# Autodesk Inventor assembly: robot_1_13
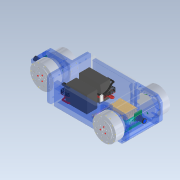
[picture p0: Inventor's stored thumbnail of the model, 180x180]
Saved by Autodesk Inventor 2020 (Build 240168000, 168)
## iProperties
Created: 2021-01-14
Part Number: robot_1_13
Document SubType Name: Assembly
Designer: DELL
Author: DELL
## Documents named in this file (19)
- F:\SoftRobot2.0\FlexipodHardware2.0\FlexipodHardware\Flexipod2.0\robot_2021_1_31\robot.iam
- F:\SoftRobot2.0\FlexipodHardware2.0\FlexipodHardware\Flexipod2.0\RMD_X6_stator.ipt
- F:\SoftRobot2.0\FlexipodHardware2.0\FlexipodHardware\Flexipod2.0\RMD_X6_rotor.ipt
- F:\SoftRobot2.0\FlexipodHardware2.0\FlexipodHardware\Flexipod2.0\Jetson nano v2- Inventor\Jetson_Nano_Dev_Kit_3D_b01.iam
- F:\SoftRobot2.0\FlexipodHardware2.0\FlexipodHardware\Flexipod2.0\battery_6s_1550_ovonic.ipt
- F:\SoftRobot2.0\FlexipodHardware2.0\FlexipodHardware\Flexipod2.0\Arducam Camera.ipt
- F:\SoftRobot2.0\FlexipodHardware2.0\FlexipodHardware\Flexipod2.0\robot_2021_1_27\shank_thigh_connector.ipt
- F:\SoftRobot2.0\FlexipodHardware2.0\FlexipodHardware\Flexipod2.0\robot_2021_1_28\hip_link_front.ipt
- F:\SoftRobot2.0\FlexipodHardware2.0\FlexipodHardware\Flexipod2.0\robot_2021_1_28\thigh_link.ipt
- F:\SoftRobot2.0\FlexipodHardware2.0\FlexipodHardware\Flexipod2.0\robot_2021_1_28\thigh_link_mirror.ipt
- F:\SoftRobot2.0\FlexipodHardware2.0\FlexipodHardware\Flexipod2.0\robot_2021_1_28\hip_link_front_mirror.ipt
- F:\SoftRobot2.0\FlexipodHardware2.0\FlexipodHardware\Flexipod2.0\robot_2021_1_28\shank_link_2.ipt
- F:\SoftRobot2.0\FlexipodHardware2.0\FlexipodHardware\Flexipod2.0\robot_2021_1_28\hip_back_motor_protector.ipt
- F:\SoftRobot2.0\FlexipodHardware2.0\FlexipodHardware\Flexipod2.0\robot_2021_1_28\hard_back_hip_2.ipt
- F:\SoftRobot2.0\FlexipodHardware2.0\FlexipodHardware\Flexipod2.0\robot_2021_1_28\hard_back_hip_2_mirror.ipt
- F:\SoftRobot2.0\FlexipodHardware2.0\FlexipodHardware\Flexipod2.0\robot_2021_1_31\back_motor_fix_board.ipt
- F:\SoftRobot2.0\FlexipodHardware2.0\FlexipodHardware\Flexipod2.0\robot_2021_1_31\buttom_camera_fix.ipt
- F:\SoftRobot2.0\FlexipodHardware2.0\FlexipodHardware\Flexipod2.0\robot_2021_1_28\body_soft2.ipt
- F:\SoftRobot2.0\FlexipodHardware2.0\FlexipodHardware\Flexipod2.0\robot_2021_1_28\body_soft2_2.ipt
## Components (55 placed, 18 different names)
1. RMD_X6_stator:1 — Mate:1, Flush:4, Mate:251, Mate:298, Mate:299
2. RMD_X6_rotor:1 — Mate:1, Flush:4, Mate:252, Mate:253
3. RMD_X6_stator:2 — Angle:2, Mate:254, Mate:255, Mate:256, Mate:257
4. RMD_X6_rotor:2 — Mate:247, Mate:248
5. RMD_X6_stator:3 — Mate:19, Mate:244, Mate:245, Mate:246
6. RMD_X6_rotor:3 — Mate:18, Mate:20
7. shank_thigh_connector:9 — Mate:18, Mate:19, Mate:20, Mate:262, Mate:263
8. RMD_X6_stator:4 — Mate:284, Mate:289, Mate:291
9. RMD_X6_rotor:4 — Mate:283, Mate:285
10. RMD_X6_stator:6 — Mate:44, Mate:231, Mate:232, Mate:233
11. RMD_X6_rotor:6 — Mate:42, Mate:43
12. shank_thigh_connector:10 — Mate:42, Mate:43, Mate:44, Mate:260, Mate:261
13. RMD_X6_rotor:7 — Flush:11, Mate:52, Mate:223, Mate:225
14. RMD_X6_stator:7 — Flush:11, Mate:52, Mate:56, Mate:57, Mate:58, Mate:224
15. RMD_X6_rotor:8 — Mate:51, Flush:10, Mate:53, Mate:54
16. RMD_X6_stator:8 — Mate:51, Flush:10, Mate:55, Mate:297, Mate:300
17. hip_link_front:1 — Mate:53, Mate:54, Mate:55, Mate:56, Mate:57, Mate:58
18. RMD_X6_rotor:9 — Mate:72, Mate:73
19. RMD_X6_stator:9 — Mate:74, Mate:228, Mate:229, Mate:230
20. RMD_X6_rotor:10 — Mate:276, Mate:278
21. RMD_X6_stator:10 — Mate:277, Mate:290, Mate:292
22. shank_thigh_connector:11 — Mate:72, Mate:73, Mate:74, Mate:264, Mate:265
23. Jetson_Nano_Dev_Kit_3D_b01:1 [sub-assembly]
24. battery_6s_1550_ovonic:1
25. battery_6s_1550_ovonic:2
26. Arducam Camera:1
27. Arducam Camera:2 — Angle:13, Mate:295, Flush:30
28. shank_link_2:3 — Mate:262, Mate:263
29. shank_link_2:4 — Mate:264, Mate:265
30. shank_link_2:2 — Mate:260, Mate:261
31. RMD_X6_rotor:13
32. RMD_X6_stator:13 — Mate:219, Mate:220, Mate:221
33. shank_thigh_connector:13 — Mate:258, Mate:259
34. shank_link_2:1 — Mate:258, Mate:259
35. RMD_X6_rotor:16 — Mate:215, Mate:216
36. RMD_X6_stator:16 — Mate:217, Mate:274, Mate:275, Mate:279
37. RMD_X6_stator:17 — Mate:236, Mate:266, Mate:267, Mate:268
38. RMD_X6_rotor:17 — Mate:237, Mate:238
39. shank_thigh_connector:14 — Mate:215, Mate:216, Mate:217, Mate:218, Mate:222
40. thigh_link:1 — Mate:218, Mate:219, Mate:220, Mate:221, Mate:222
41. shank_thigh_connector:15 — Mate:223, Mate:224, Mate:225, Mate:226, Mate:227
42. thigh_link:2 — Mate:226, Mate:227, Mate:228, Mate:229, Mate:230
43. thigh_link_mirror:1 — Mate:231, Mate:232, Mate:233, Mate:234, Mate:235
44. shank_thigh_connector:16 — Mate:234, Mate:235, Mate:236, Mate:237, Mate:238
45. thigh_link:3 — Mate:244, Mate:245, Mate:246, Mate:249, Mate:250
46. shank_thigh_connector:17 — Mate:247, Mate:248, Mate:249, Mate:250, Mate:257
47. hip_link_front_mirror:1 — Mate:251, Mate:252, Mate:253, Mate:254, Mate:255, Mate:256
48. hip_back_motor_protector:1 — Mate:266, Mate:267, Mate:268, Mate:286, Mate:287, Mate:288
49. hip_back_motor_protector:2 — Mate:274, Mate:275, Mate:279, Mate:280, Mate:281, Mate:282
50. hard_back_hip_2:1 — Mate:283, Mate:284, Mate:285, Mate:286, Mate:287, Mate:288
51. hard_back_hip_2_mirror:1 — Mate:276, Mate:277, Mate:278, Mate:280, Mate:281, Mate:282
52. back_motor_fix_board:1 — Angle:13, Mate:289, Mate:290, Mate:291, Mate:292, Mate:293, Flush:26, Flush:27, Mate:296, Flush:34, Flush:36
53. buttom_camera_fix:1 — Mate:293, Flush:26, Flush:27, Mate:295, Flush:30
54. body_soft2:1 — Flush:31, Flush:33, Mate:296, Flush:34, Flush:35, Mate:297, Mate:298, Mate:299, Mate:300, Flush:36, Mate:301, Flush:37, Tangent:1
55. body_soft2_2:1 — Mate:301, Flush:37, Tangent:1
## Relationships (130: Mate 106, Flush 21, Angle 2, Tangent 1)
- Mate:1: RMD_X6_stator:1 ↔ RMD_X6_rotor:1
- Flush:4 (-3 mm): RMD_X6_stator:1 ↔ RMD_X6_rotor:1
- [Mate]: RMD_X6_stator:2 ↔ RMD_X6_rotor:2
- [Flush] (-3 mm): RMD_X6_stator:2 ↔ RMD_X6_rotor:2
- [Mate]: RMD_X6_stator:3 ↔ RMD_X6_rotor:3
- [Flush] (-3 mm): RMD_X6_stator:3 ↔ RMD_X6_rotor:3
- Angle:2 (180 deg): RMD_X6_stator:2
- Mate:18: RMD_X6_rotor:3 ↔ shank_thigh_connector:9
- Mate:19: RMD_X6_stator:3 ↔ shank_thigh_connector:9
- Mate:20: RMD_X6_rotor:3 ↔ shank_thigh_connector:9
- [Mate]: RMD_X6_stator:4 ↔ RMD_X6_rotor:4
- [Flush] (-3 mm): RMD_X6_stator:4 ↔ RMD_X6_rotor:4
- [Mate]: RMD_X6_stator:6 ↔ RMD_X6_rotor:6
- [Flush] (-3 mm): RMD_X6_stator:6 ↔ RMD_X6_rotor:6
- Mate:42: RMD_X6_rotor:6 ↔ shank_thigh_connector:10
- Mate:43: RMD_X6_rotor:6 ↔ shank_thigh_connector:10
- Mate:44: RMD_X6_stator:6 ↔ shank_thigh_connector:10
- Mate:51: RMD_X6_rotor:8 ↔ RMD_X6_stator:8
- Flush:10 (-3 mm): RMD_X6_rotor:8 ↔ RMD_X6_stator:8
- Flush:11 (-3 mm): RMD_X6_rotor:7 ↔ RMD_X6_stator:7
- Mate:52: RMD_X6_rotor:7 ↔ RMD_X6_stator:7
- Mate:53: RMD_X6_rotor:8 ↔ hip_link_front:1
- Mate:54: RMD_X6_rotor:8 ↔ hip_link_front:1
- Mate:55: RMD_X6_stator:8 ↔ hip_link_front:1
- Mate:56: RMD_X6_stator:7 ↔ hip_link_front:1
- Mate:57: RMD_X6_stator:7 ↔ hip_link_front:1
- Mate:58: RMD_X6_stator:7 ↔ hip_link_front:1
- [Mate]: RMD_X6_rotor:9 ↔ RMD_X6_stator:9
- [Flush] (-3 mm): RMD_X6_rotor:9 ↔ RMD_X6_stator:9
- [Mate]: RMD_X6_rotor:10 ↔ RMD_X6_stator:10
- [Flush] (-3 mm): RMD_X6_rotor:10 ↔ RMD_X6_stator:10
- Mate:72: RMD_X6_rotor:9 ↔ shank_thigh_connector:11
- Mate:73: RMD_X6_rotor:9 ↔ shank_thigh_connector:11
- Mate:74: RMD_X6_stator:9 ↔ shank_thigh_connector:11
- [Mate]: RMD_X6_rotor:13 ↔ RMD_X6_stator:13
- [Flush] (-3 mm): RMD_X6_rotor:13 ↔ RMD_X6_stator:13
- [Mate]: RMD_X6_rotor:13 ↔ shank_thigh_connector:13
- [Mate]: RMD_X6_rotor:13 ↔ shank_thigh_connector:13
- [Mate]: RMD_X6_stator:13 ↔ shank_thigh_connector:13
- [Flush] (-3 mm): RMD_X6_rotor:16 ↔ RMD_X6_stator:16
- [Mate]: RMD_X6_rotor:16 ↔ RMD_X6_stator:16
- [Mate]: RMD_X6_stator:17 ↔ RMD_X6_rotor:17
- [Flush] (-3 mm): RMD_X6_stator:17 ↔ RMD_X6_rotor:17
- Mate:215: RMD_X6_rotor:16 ↔ shank_thigh_connector:14
- Mate:216: RMD_X6_rotor:16 ↔ shank_thigh_connector:14
- Mate:217: RMD_X6_stator:16 ↔ shank_thigh_connector:14
- Mate:218: shank_thigh_connector:14 ↔ thigh_link:1
- Mate:219: RMD_X6_stator:13 ↔ thigh_link:1
- Mate:220: RMD_X6_stator:13 ↔ thigh_link:1
- Mate:221: RMD_X6_stator:13 ↔ thigh_link:1
- Mate:222: shank_thigh_connector:14 ↔ thigh_link:1
- Mate:223: RMD_X6_rotor:7 ↔ shank_thigh_connector:15
- Mate:224: RMD_X6_stator:7 ↔ shank_thigh_connector:15
- Mate:225: RMD_X6_rotor:7 ↔ shank_thigh_connector:15
- Mate:226: shank_thigh_connector:15 ↔ thigh_link:2
- Mate:227: shank_thigh_connector:15 ↔ thigh_link:2
- Mate:228: RMD_X6_stator:9 ↔ thigh_link:2
- Mate:229: RMD_X6_stator:9 ↔ thigh_link:2
- Mate:230: RMD_X6_stator:9 ↔ thigh_link:2
- Mate:231: RMD_X6_stator:6 ↔ thigh_link_mirror:1
- Mate:232: RMD_X6_stator:6 ↔ thigh_link_mirror:1
- Mate:233: RMD_X6_stator:6 ↔ thigh_link_mirror:1
- Mate:234: thigh_link_mirror:1 ↔ shank_thigh_connector:16
- Mate:235: thigh_link_mirror:1 ↔ shank_thigh_connector:16
- Mate:236: RMD_X6_stator:17 ↔ shank_thigh_connector:16
- Mate:237: RMD_X6_rotor:17 ↔ shank_thigh_connector:16
- Mate:238: RMD_X6_rotor:17 ↔ shank_thigh_connector:16
- Mate:244: RMD_X6_stator:3 ↔ thigh_link:3
- Mate:245: RMD_X6_stator:3 ↔ thigh_link:3
- Mate:246: RMD_X6_stator:3 ↔ thigh_link:3
- Mate:247: RMD_X6_rotor:2 ↔ shank_thigh_connector:17
- Mate:248: RMD_X6_rotor:2 ↔ shank_thigh_connector:17
- Mate:249: thigh_link:3 ↔ shank_thigh_connector:17
- Mate:250: thigh_link:3 ↔ shank_thigh_connector:17
- Mate:251: RMD_X6_stator:1 ↔ hip_link_front_mirror:1
- Mate:252: RMD_X6_rotor:1 ↔ hip_link_front_mirror:1
- Mate:253: RMD_X6_rotor:1 ↔ hip_link_front_mirror:1
- Mate:254: RMD_X6_stator:2 ↔ hip_link_front_mirror:1
- Mate:255: RMD_X6_stator:2 ↔ hip_link_front_mirror:1
- Mate:256: RMD_X6_stator:2 ↔ hip_link_front_mirror:1
- Mate:257: RMD_X6_stator:2 ↔ shank_thigh_connector:17
- Mate:258: shank_thigh_connector:13 ↔ shank_link_2:1
- Mate:259: shank_thigh_connector:13 ↔ shank_link_2:1
- Mate:260: shank_thigh_connector:10 ↔ shank_link_2:2
- Mate:261: shank_thigh_connector:10 ↔ shank_link_2:2
- Mate:262: shank_thigh_connector:9 ↔ shank_link_2:3
- Mate:263: shank_thigh_connector:9 ↔ shank_link_2:3
- Mate:264: shank_thigh_connector:11 ↔ shank_link_2:4
- Mate:265: shank_thigh_connector:11 ↔ shank_link_2:4
- Mate:266: RMD_X6_stator:17 ↔ hip_back_motor_protector:1
- Mate:267: RMD_X6_stator:17 ↔ hip_back_motor_protector:1
- Mate:268: RMD_X6_stator:17 ↔ hip_back_motor_protector:1
- Mate:274: RMD_X6_stator:16 ↔ hip_back_motor_protector:2
- Mate:275: RMD_X6_stator:16 ↔ hip_back_motor_protector:2
- Mate:276: RMD_X6_rotor:10 ↔ hard_back_hip_2_mirror:1
- Mate:277: RMD_X6_stator:10 ↔ hard_back_hip_2_mirror:1
- Mate:278: RMD_X6_rotor:10 ↔ hard_back_hip_2_mirror:1
- Mate:279: RMD_X6_stator:16 ↔ hip_back_motor_protector:2
- Mate:280: hip_back_motor_protector:2 ↔ hard_back_hip_2_mirror:1
- Mate:281: hip_back_motor_protector:2 ↔ hard_back_hip_2_mirror:1
- Mate:282: hip_back_motor_protector:2 ↔ hard_back_hip_2_mirror:1
- Mate:283: RMD_X6_rotor:4 ↔ hard_back_hip_2:1
- Mate:284: RMD_X6_stator:4 ↔ hard_back_hip_2:1
- Mate:285: RMD_X6_rotor:4 ↔ hard_back_hip_2:1
- Mate:286: hip_back_motor_protector:1 ↔ hard_back_hip_2:1
- Mate:287: hip_back_motor_protector:1 ↔ hard_back_hip_2:1
- Mate:288: hip_back_motor_protector:1 ↔ hard_back_hip_2:1
- Angle:13 (0 deg): Arducam Camera:2 ↔ back_motor_fix_board:1
- Mate:289: RMD_X6_stator:4 ↔ back_motor_fix_board:1
- Mate:290: RMD_X6_stator:10 ↔ back_motor_fix_board:1
- Mate:291: RMD_X6_stator:4 ↔ back_motor_fix_board:1
- Mate:292: RMD_X6_stator:10 ↔ back_motor_fix_board:1
- Mate:293: back_motor_fix_board:1 ↔ buttom_camera_fix:1
- Flush:26: back_motor_fix_board:1 ↔ buttom_camera_fix:1
- Flush:27: back_motor_fix_board:1 ↔ buttom_camera_fix:1
- Mate:295: Arducam Camera:2 ↔ buttom_camera_fix:1
- Flush:30: Arducam Camera:2 ↔ buttom_camera_fix:1
- Flush:31: body_soft2:1
- Flush:33: body_soft2:1
- Mate:296: back_motor_fix_board:1 ↔ body_soft2:1
- Flush:34: back_motor_fix_board:1 ↔ body_soft2:1
- Flush:35: body_soft2:1
- Mate:297: RMD_X6_stator:8 ↔ body_soft2:1
- Mate:298: RMD_X6_stator:1 ↔ body_soft2:1
- Mate:299: RMD_X6_stator:1 ↔ body_soft2:1
- Mate:300: RMD_X6_stator:8 ↔ body_soft2:1
- Flush:36: back_motor_fix_board:1 ↔ body_soft2:1
- Mate:301: body_soft2:1 ↔ body_soft2_2:1
- Flush:37: body_soft2:1 ↔ body_soft2_2:1
- Tangent:1: body_soft2:1 ↔ body_soft2_2:1
## Named parameters: d11_d3 = 0 mm, d12_d4 = -3 mm, d13_d3 = 0 mm, d14_d4 = -3 mm, d32_d13_d3 = 0 mm, d33_d14_d4 = -3 mm, d36_d13_d3 = 0 mm, d37_d14_d4 = -3 mm, d79_d64 = 0 mm, d80_d65 = -3 mm, d81_d64 = 0 mm, d82_d65 = -3 mm, d241_d93 = 0 mm, d242_d94 = 0 mm, d243_d95 = 0 mm, d244_d79_d64 = 0 mm, d245_d80_d65 = -3 mm, d258_d66 = -3 mm, d259_d67 = 0 mm, d260_d11_d3 = 0 mm, d261_d12_d4 = -3 mm
